# Autodesk Inventor assembly: X Axis
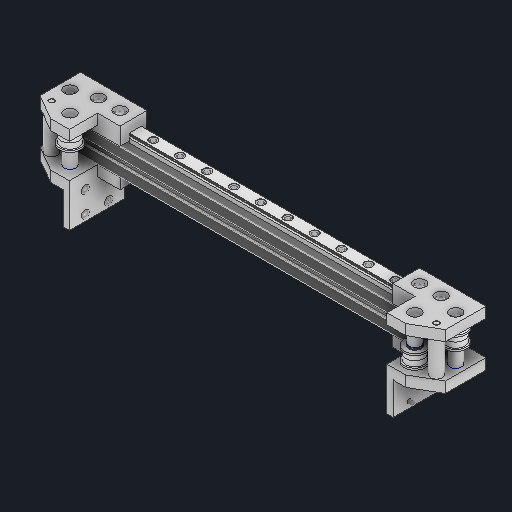
[picture p0: Inventor's stored thumbnail of the model, 512x512]
Saved by Autodesk Inventor 2025.1 (Build 291241020, 241B)
## iProperties
Created: 2025-05-09
Part Number: X Axis
Document SubType Name: Assembly
Designer: AdminForWorker
Title: X Axis
Author: AdminForWorker
## Documents named in this file (6)
- C:\Users\Joshua Eah\Documents\Voron 0.2\CAD\Master Assembly\X Axis.iam
- C:\Users\Joshua Eah\Documents\Voron 0.2\CAD\Master Assembly\XY Joint Left.iam
- C:\Users\Joshua Eah\Documents\Voron 0.2\CAD\Master Assembly\XY Joint Right.iam
- C:\Users\Joshua Eah\Documents\Voron 0.2\CAD\Master Assembly\Linear Rail\MGN7 Rail 150mm.iam
- MGN7 150mm Rail.iam
- C:\Users\Joshua Eah\Documents\Voron 0.2\CAD\Master Assembly\Frame\Parts\Extrusions\1515 200mm - A.ipt
## Components (4 placed, 4 different names)
1. XY Joint Left:1 [sub-assembly]
2. XY Joint Right:1 [sub-assembly] — Mate:3
3. MGN7 150mm Rail:1 [sub-assembly] — Mate:1, Mate:2, Mate:3
4. 1515 200mm - A (1):1 — Mate:1, Mate:2
## Relationships (3: Mate 3)
- Mate:1 (0.1 mm): MGN7 150mm Rail:1 ↔ 1515 200mm - A (1):1
- Mate:2: MGN7 150mm Rail:1 ↔ 1515 200mm - A (1):1
- Mate:3 (1 mm): XY Joint Right:1 ↔ MGN7 150mm Rail:1
